# Autodesk Inventor assembly: Assembly
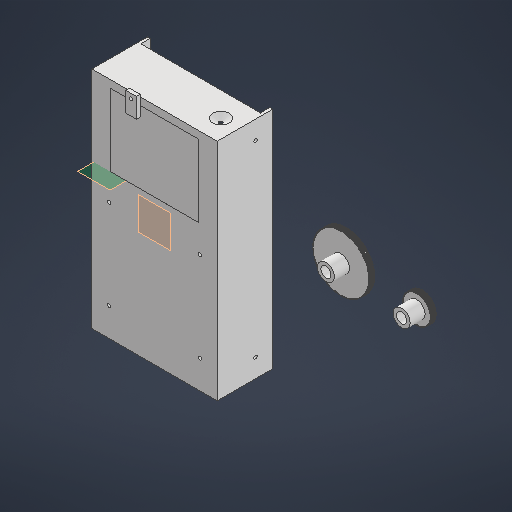
[picture p0: Inventor's stored thumbnail of the model, 512x512]
Saved by Autodesk Inventor 2027 (Build 310192000, 192)
## iProperties
Created: 2026-03-08
Part Number: Assembly
Document SubType Name: Assembly
Designer: kjedr
Author: kjedr
## Documents named in this file (5)
- C:\Users\kjedr\Documents\GitHub\ECE445-UIUC-Heterodyne\Chassis\Assembly.iam
- C:\Users\kjedr\Documents\GitHub\ECE445-UIUC-Heterodyne\Chassis\Bottom_Shell.ipt
- C:\Users\kjedr\Documents\GitHub\ECE445-UIUC-Heterodyne\Chassis\Dial.ipt
- C:\Users\kjedr\Documents\GitHub\ECE445-UIUC-Heterodyne\Chassis\freqDial1.ipt
- C:\Users\kjedr\Documents\GitHub\ECE445-UIUC-Heterodyne\Chassis\batteryFlap.ipt
## Components (4 placed, 4 different names)
1. Bottom_Shell:1 — Flush:1, Mate:1, Mate:2
2. Dial:2
3. freqDial1:1
4. batteryFlap:1 — Flush:1, Mate:1, Mate:2
## Relationships (3: Mate 2, Flush 1)
- Flush:1: Bottom_Shell:1 ↔ batteryFlap:1
- Mate:1: Bottom_Shell:1 ↔ batteryFlap:1
- Mate:2: Bottom_Shell:1 ↔ batteryFlap:1
